# Autodesk Inventor assembly: Assembly1
(part 7 of 8)
## Named parameters: d38_d13 = 0 mm, d39_d14 = 0 mm, d40_d15 = 270 deg, d41_d16 = 0 mm, d42_d17 = 270 deg, d43_d3 = 25 deg, d44_d4 = -25 deg, d45_d5 = 25 deg, d46_d6 = -25 deg, d47_d2 = 0 mm, d48_d30 = 0 mm, d58_d13 = 0 mm, d59_d14 = 0 mm, d60_d15 = 270 deg, d61_d16 = 0 mm, d62_d17 = 270 deg, d63_d3 = 25 deg, d64_d4 = -25 deg, d65_d5 = 25 deg, d66_d6 = -25 deg, d67_d2 = 0 mm, d68_d30 = 0 mm, d78_d13 = 0 mm, d79_d14 = 0 mm, d80_d15 = 270 deg, d81_d16 = 0 mm, d82_d17 = 270 deg, d83_d3 = 25 deg, d84_d4 = -25 deg, d85_d5 = 25 deg, d86_d6 = -25 deg, d87_d2 = 0 mm, d88_d30 = 0 mm, d95_d13 = 0 mm, d96_d14 = 0 mm, d97_d15 = 270 deg, d98_d16 = 0 mm, d99_d17 = 270 deg, d100_d3 = 25 deg, d101_d4 = -25 deg, d102_d5 = 25 deg, d103_d6 = -25 deg, d104_d2 = 0 mm, d105_d30 = 0 mm, d112_d13 = 0 mm, d113_d14 = 0 mm, d114_d15 = 270 deg, d115_d16 = 0 mm, d116_d17 = 270 deg, d117_d3 = 25 deg, d118_d4 = -25 deg, d119_d5 = 25 deg, d120_d6 = -25 deg, d121_d2 = 0 mm, d122_d30 = 0 mm, d129_d13 = 0 mm, d130_d14 = 0 mm, d131_d15 = 270 deg, d132_d16 = 0 mm, d133_d17 = 270 deg, d134_d3 = 25 deg, d135_d4 = -25 deg, d136_d5 = 25 deg, d137_d6 = -25 deg, d138_d2 = 0 mm, d139_d30 = 0 mm, d146_d13 = 0 mm, d147_d14 = 0 mm, d148_d15 = 270 deg, d149_d16 = 0 mm, d150_d17 = 270 deg, d151_d3 = 25 deg, d152_d4 = -25 deg, d153_d5 = 25 deg, d154_d6 = -25 deg, d155_d2 = 0 mm, d156_d30 = 0 mm, d163_d13 = 0 mm, d164_d14 = 0 mm, d165_d15 = 270 deg, d166_d16 = 0 mm, d167_d17 = 270 deg, d168_d3 = 25 deg, d169_d4 = -25 deg, d170_d5 = 25 deg, d171_d6 = -25 deg, d172_d2 = 0 mm, d173_d30 = 0 mm, d180_d13 = 0 mm, d181_d14 = 0 mm, d182_d15 = 270 deg, d183_d16 = 0 mm, d184_d17 = 270 deg, d185_d3 = 25 deg, d186_d4 = -25 deg, d187_d5 = 25 deg, d188_d6 = -25 deg, d189_d2 = 0 mm, d190_d30 = 0 mm, d197_d13 = 0 mm, d198_d14 = 0 mm, d199_d15 = 270 deg, d200_d16 = 0 mm, d201_d17 = 270 deg, d202_d3 = 25 deg, d203_d4 = -25 deg, d204_d5 = 25 deg, d205_d6 = -25 deg, d206_d2 = 0 mm, d207_d30 = 0 mm, d214_d13 = 0 mm, d215_d14 = 0 mm, d216_d15 = 270 deg, d217_d16 = 0 mm, d218_d17 = 270 deg, d219_d3 = 25 deg, d220_d4 = -25 deg, d221_d5 = 25 deg, d222_d6 = -25 deg, d223_d2 = 0 mm, d224_d30 = 0 mm, d231_d13 = 0 mm, d232_d14 = 0 mm, d233_d15 = 270 deg, d234_d16 = 0 mm, d235_d17 = 270 deg, d236_d3 = 25 deg, d237_d4 = -25 deg, d238_d5 = 25 deg, d239_d6 = -25 deg, d240_d2 = 0 mm, d241_d30 = 0 mm, d248_d13 = 0 mm, d249_d14 = 0 mm, d250_d15 = 270 deg, d251_d16 = 0 mm, d252_d17 = 270 deg, d253_d3 = 25 deg, d254_d4 = -25 deg, d255_d5 = 25 deg, d256_d6 = -25 deg, d257_d2 = 0 mm, d258_d30 = 0 mm, d265_d13 = 0 mm, d266_d14 = 0 mm, d267_d15 = 270 deg, d268_d16 = 0 mm, d269_d17 = 270 deg, d270_d3 = 25 deg, d271_d4 = -25 deg, d272_d5 = 25 deg, d273_d6 = -25 deg, d274_d2 = 0 mm, d275_d30 = 0 mm, d318_d248_d13 = 0 mm, d319_d249_d14 = 0 mm, d320_d250_d15 = 270 deg, d321_d251_d16 = 0 mm, d322_d252_d17 = 270 deg, d323_d253_d3 = 25 deg, d324_d254_d4 = -25 deg, d325_d255_d5 = 25 deg, d326_d256_d6 = -25 deg, d327_d257_d2 = 0 mm, d328_d258_d30 = 0 mm, d335_d248_d13 = 0 mm, d336_d249_d14 = 0 mm, d337_d250_d15 = 270 deg, d338_d251_d16 = 0 mm, d339_d252_d17 = 270 deg, d340_d253_d3 = 25 deg, d341_d254_d4 = -25 deg, d342_d255_d5 = 25 deg, d343_d256_d6 = -25 deg, d344_d257_d2 = 0 mm, d345_d258_d30 = 0 mm, d352_d248_d13 = 0 mm, d353_d249_d14 = 0 mm, d354_d250_d15 = 270 deg, d355_d251_d16 = 0 mm, d356_d252_d17 = 270 deg, d357_d253_d3 = 25 deg, d358_d254_d4 = -25 deg, d359_d255_d5 = 25 deg, d360_d256_d6 = -25 deg, d361_d257_d2 = 0 mm, d362_d258_d30 = 0 mm, d369_d248_d13 = 0 mm, d370_d249_d14 = 0 mm, d371_d250_d15 = 270 deg, d372_d251_d16 = 0 mm, d373_d252_d17 = 270 deg, d374_d253_d3 = 25 deg, d375_d254_d4 = -25 deg, d376_d255_d5 = 25 deg, d377_d256_d6 = -25 deg, d378_d257_d2 = 0 mm, d379_d258_d30 = 0 mm, d386_d248_d13 = 0 mm, d387_d249_d14 = 0 mm, d388_d250_d15 = 270 deg, d389_d251_d16 = 0 mm, d390_d252_d17 = 270 deg, d391_d253_d3 = 25 deg, d392_d254_d4 = -25 deg, d393_d255_d5 = 25 deg, d394_d256_d6 = -25 deg, d395_d257_d2 = 0 mm, d396_d258_d30 = 0 mm, d418_d248_d13 = 0 mm, d419_d249_d14 = 0 mm, d420_d250_d15 = 270 deg, d421_d251_d16 = 0 mm, d422_d252_d17 = 270 deg, d423_d253_d3 = 25 deg, d424_d254_d4 = -25 deg, d425_d255_d5 = 25 deg, d426_d256_d6 = -25 deg, d427_d257_d2 = 0 mm, d428_d258_d30 = 0 mm, d435_d248_d13 = 0 mm, d436_d249_d14 = 0 mm, d437_d250_d15 = 270 deg, d438_d251_d16 = 0 mm, d439_d252_d17 = 270 deg, d440_d253_d3 = 25 deg, d441_d254_d4 = -25 deg, d442_d255_d5 = 25 deg, d443_d256_d6 = -25 deg, d444_d257_d2 = 0 mm, d445_d258_d30 = 0 mm, d452_d248_d13 = 0 mm, d453_d249_d14 = 0 mm, d454_d250_d15 = 270 deg, d455_d251_d16 = 0 mm, d456_d252_d17 = 270 deg, d457_d253_d3 = 25 deg, d458_d254_d4 = -25 deg, d459_d255_d5 = 25 deg, d460_d256_d6 = -25 deg, d461_d257_d2 = 0 mm, d462_d258_d30 = 0 mm, d469_d248_d13 = 0 mm, d470_d249_d14 = 0 mm, d471_d250_d15 = 270 deg, d472_d251_d16 = 0 mm, d473_d252_d17 = 270 deg, d474_d253_d3 = 25 deg, d475_d254_d4 = -25 deg, d476_d255_d5 = 25 deg, d477_d256_d6 = -25 deg, d478_d257_d2 = 0 mm, d479_d258_d30 = 0 mm, d498_d248_d13 = 0 mm, d499_d249_d14 = 0 mm, d500_d250_d15 = 270 deg, d501_d251_d16 = 0 mm, d502_d252_d17 = 270 deg, d503_d253_d3 = 25 deg, d504_d254_d4 = -25 deg, d505_d255_d5 = 25 deg, d506_d256_d6 = -25 deg, d507_d257_d2 = 0 mm, d508_d258_d30 = 0 mm, d515_d248_d13 = 0 mm, d516_d249_d14 = 0 mm, d517_d250_d15 = 270 deg, d518_d251_d16 = 0 mm, d519_d252_d17 = 270 deg, d520_d253_d3 = 25 deg, d521_d254_d4 = -25 deg, d522_d255_d5 = 25 deg, d523_d256_d6 = -25 deg, d524_d257_d2 = 0 mm, d525_d258_d30 = 0 mm, d532_d248_d13 = 0 mm, d533_d249_d14 = 0 mm, d534_d250_d15 = 270 deg, d535_d251_d16 = 0 mm, d536_d252_d17 = 270 deg, d537_d253_d3 = 25 deg, d538_d254_d4 = -25 deg, d539_d255_d5 = 25 deg, d540_d256_d6 = -25 deg, d541_d257_d2 = 0 mm, d542_d258_d30 = 0 mm, d549_d248_d13 = 0 mm, d550_d249_d14 = 0 mm, d551_d250_d15 = 270 deg, d552_d251_d16 = 0 mm, d553_d252_d17 = 270 deg, d554_d253_d3 = 25 deg, d555_d254_d4 = -25 deg, d556_d255_d5 = 25 deg, d557_d256_d6 = -25 deg, d558_d257_d2 = 0 mm, d559_d258_d30 = 0 mm, d566_d248_d13 = 0 mm, d567_d249_d14 = 0 mm, d568_d250_d15 = 270 deg, d569_d251_d16 = 0 mm, d570_d252_d17 = 270 deg, d571_d253_d3 = 25 deg, d572_d254_d4 = -25 deg, d573_d255_d5 = 25 deg, d574_d256_d6 = -25 deg, d575_d257_d2 = 0 mm, d576_d258_d30 = 0 mm, d583_d248_d13 = 0 mm, d584_d249_d14 = 0 mm, d585_d250_d15 = 270 deg, d586_d251_d16 = 0 mm, d587_d252_d17 = 270 deg, d588_d253_d3 = 25 deg, d589_d254_d4 = -25 deg, d590_d255_d5 = 25 deg, d591_d256_d6 = -25 deg, d592_d257_d2 = 0 mm, d593_d258_d30 = 0 mm, d600_d248_d13 = 0 mm, d601_d249_d14 = 0 mm, d602_d250_d15 = 270 deg, d603_d251_d16 = 0 mm, d604_d252_d17 = 270 deg, d605_d253_d3 = 25 deg, d606_d254_d4 = -25 deg, d607_d255_d5 = 25 deg, d608_d256_d6 = -25 deg, d609_d257_d2 = 0 mm, d610_d258_d30 = 0 mm, d617_d248_d13 = 0 mm, d618_d249_d14 = 0 mm, d619_d250_d15 = 270 deg, d620_d251_d16 = 0 mm, d621_d252_d17 = 270 deg, d622_d253_d3 = 25 deg, d623_d254_d4 = -25 deg, d624_d255_d5 = 25 deg, d625_d256_d6 = -25 deg, d626_d257_d2 = 0 mm, d627_d258_d30 = 0 mm, d634_d248_d13 = 0 mm, d635_d249_d14 = 0 mm, d636_d250_d15 = 270 deg, d637_d251_d16 = 0 mm, d638_d252_d17 = 270 deg, d639_d253_d3 = 25 deg, d640_d254_d4 = -25 deg, d641_d255_d5 = 25 deg, d642_d256_d6 = -25 deg, d643_d257_d2 = 0 mm, d644_d258_d30 = 0 mm, d651_d248_d13 = 0 mm, d652_d249_d14 = 0 mm, d653_d250_d15 = 270 deg, d654_d251_d16 = 0 mm, d655_d252_d17 = 270 deg, d656_d253_d3 = 25 deg, d657_d254_d4 = -25 deg, d658_d255_d5 = 25 deg, d659_d256_d6 = -25 deg, d660_d257_d2 = 0 mm, d661_d258_d30 = 0 mm, d668_d248_d13 = 0 mm, d669_d249_d14 = 0 mm, d670_d250_d15 = 270 deg, d671_d251_d16 = 0 mm, d672_d252_d17 = 270 deg, d673_d253_d3 = 25 deg, d674_d254_d4 = -25 deg, d675_d255_d5 = 25 deg, d676_d256_d6 = -25 deg, d677_d257_d2 = 0 mm, d678_d258_d30 = 0 mm, d685_d248_d13 = 0 mm, d686_d249_d14 = 0 mm, d687_d250_d15 = 270 deg, d688_d251_d16 = 0 mm, d689_d252_d17 = 270 deg, d690_d253_d3 = 25 deg, d691_d254_d4 = -25 deg, d692_d255_d5 = 25 deg, d693_d256_d6 = -25 deg, d694_d257_d2 = 0 mm, d695_d258_d30 = 0 mm, d702_d248_d13 = 0 mm, d703_d249_d14 = 0 mm, d704_d250_d15 = 270 deg, d705_d251_d16 = 0 mm, d706_d252_d17 = 270 deg, d707_d253_d3 = 25 deg, d708_d254_d4 = -25 deg, d709_d255_d5 = 25 deg, d710_d256_d6 = -25 deg, d711_d257_d2 = 0 mm, d712_d258_d30 = 0 mm, d758_d248_d13 = 0 mm, d759_d249_d14 = 0 mm, d760_d250_d15 = 270 deg, d761_d251_d16 = 0 mm, d762_d252_d17 = 270 deg, d763_d253_d3 = 25 deg, d764_d254_d4 = -25 deg, d765_d255_d5 = 25 deg, d766_d256_d6 = -25 deg, d767_d257_d2 = 0 mm, d768_d258_d30 = 0 mm, d775_d248_d13 = 0 mm, d776_d249_d14 = 0 mm, d777_d250_d15 = 270 deg, d778_d251_d16 = 0 mm, d779_d252_d17 = 270 deg, d780_d253_d3 = 25 deg, d781_d254_d4 = -25 deg, d782_d255_d5 = 25 deg, d783_d256_d6 = -25 deg, d784_d257_d2 = 0 mm, d785_d258_d30 = 0 mm, d792_d248_d13 = 0 mm, d793_d249_d14 = 0 mm, d794_d250_d15 = 270 deg, d795_d251_d16 = 0 mm, d796_d252_d17 = 270 deg, d797_d253_d3 = 25 deg, d798_d254_d4 = -25 deg, d799_d255_d5 = 25 deg, d800_d256_d6 = -25 deg, d801_d257_d2 = 0 mm, d802_d258_d30 = 0 mm, d809_d248_d13 = 0 mm, d810_d249_d14 = 0 mm, d811_d250_d15 = 270 deg, d812_d251_d16 = 0 mm, d813_d252_d17 = 270 deg, d814_d253_d3 = 25 deg, d815_d254_d4 = -25 deg, d816_d255_d5 = 25 deg, d817_d256_d6 = -25 deg, d818_d257_d2 = 0 mm, d819_d258_d30 = 0 mm, d826_d248_d13 = 0 mm, d827_d249_d14 = 0 mm, d828_d250_d15 = 270 deg, d829_d251_d16 = 0 mm, d830_d252_d17 = 270 deg, d831_d253_d3 = 25 deg, d832_d254_d4 = -25 deg, d833_d255_d5 = 25 deg, d834_d256_d6 = -25 deg, d835_d257_d2 = 0 mm, d836_d258_d30 = 0 mm, d843_d248_d13 = 0 mm, d844_d249_d14 = 0 mm, d845_d250_d15 = 270 deg, d846_d251_d16 = 0 mm, d847_d252_d17 = 270 deg, d848_d253_d3 = 25 deg, d849_d254_d4 = -25 deg, d850_d255_d5 = 25 deg, d851_d256_d6 = -25 deg, d852_d257_d2 = 0 mm, d853_d258_d30 = 0 mm, d860_d248_d13 = 0 mm, d861_d249_d14 = 0 mm, d862_d250_d15 = 270 deg, d863_d251_d16 = 0 mm, d864_d252_d17 = 270 deg, d865_d253_d3 = 25 deg, d866_d254_d4 = -25 deg, d867_d255_d5 = 25 deg, d868_d256_d6 = -25 deg, d869_d257_d2 = 0 mm, d870_d258_d30 = 0 mm, d877_d248_d13 = 0 mm, d878_d249_d14 = 0 mm, d879_d250_d15 = 270 deg, d880_d251_d16 = 0 mm, d881_d252_d17 = 270 deg, d882_d253_d3 = 25 deg, d883_d254_d4 = -25 deg, d884_d255_d5 = 25 deg, d885_d256_d6 = -25 deg, d886_d257_d2 = 0 mm, d887_d258_d30 = 0 mm, d918_d248_d13 = 0 mm, d919_d249_d14 = 0 mm, d920_d250_d15 = 270 deg, d921_d251_d16 = 0 mm, d922_d252_d17 = 270 deg, d923_d253_d3 = 25 deg, d924_d254_d4 = -25 deg, d925_d255_d5 = 25 deg, d926_d256_d6 = -25 deg, d927_d257_d2 = 0 mm, d928_d258_d30 = 0 mm, d935_d248_d13 = 0 mm, d936_d249_d14 = 0 mm, d937_d250_d15 = 270 deg, d938_d251_d16 = 0 mm, d939_d252_d17 = 270 deg, d940_d253_d3 = 25 deg, d941_d254_d4 = -25 deg, d942_d255_d5 = 25 deg, d943_d256_d6 = -25 deg, d944_d257_d2 = 0 mm, d945_d258_d30 = 0 mm, d952_d248_d13 = 0 mm, d953_d249_d14 = 0 mm, d954_d250_d15 = 270 deg, d955_d251_d16 = 0 mm, d956_d252_d17 = 270 deg, d957_d253_d3 = 25 deg, d958_d254_d4 = -25 deg, d959_d255_d5 = 25 deg, d960_d256_d6 = -25 deg, d961_d257_d2 = 0 mm, d962_d258_d30 = 0 mm, d986_d248_d13 = 0 mm, d987_d249_d14 = 0 mm, d988_d250_d15 = 270 deg, d989_d251_d16 = 0 mm, d990_d252_d17 = 270 deg, d991_d253_d3 = 25 deg, d992_d254_d4 = -25 deg, d993_d255_d5 = 25 deg, d994_d256_d6 = -25 deg, d995_d257_d2 = 0 mm, d996_d258_d30 = 0 mm, d1003_d248_d13 = 0 mm, d1004_d249_d14 = 0 mm, d1005_d250_d15 = 270 deg, d1006_d251_d16 = 0 mm, d1007_d252_d17 = 270 deg, d1008_d253_d3 = 25 deg, d1009_d254_d4 = -25 deg, d1010_d255_d5 = 25 deg, d1011_d256_d6 = -25 deg, d1012_d257_d2 = 0 mm, d1013_d258_d30 = 0 mm, d1037_d248_d13 = 0 mm, d1038_d249_d14 = 0 mm, d1039_d250_d15 = 270 deg, d1040_d251_d16 = 0 mm, d1041_d252_d17 = 270 deg, d1042_d253_d3 = 25 deg, d1043_d254_d4 = -25 deg, d1044_d255_d5 = 25 deg, d1045_d256_d6 = -25 deg, d1046_d257_d2 = 0 mm, d1047_d258_d30 = 0 mm, d1071_d248_d13 = 0 mm, d1072_d249_d14 = 0 mm, d1073_d250_d15 = 270 deg, d1074_d251_d16 = 0 mm, d1075_d252_d17 = 270 deg, d1076_d253_d3 = 25 deg, d1077_d254_d4 = -25 deg, d1078_d255_d5 = 25 deg, d1079_d256_d6 = -25 deg, d1080_d257_d2 = 0 mm, d1081_d258_d30 = 0 mm, d1105_d248_d13 = 0 mm, d1106_d249_d14 = 0 mm, d1107_d250_d15 = 270 deg, d1108_d251_d16 = 0 mm, d1109_d252_d17 = 270 deg, d1110_d253_d3 = 25 deg, d1111_d254_d4 = -25 deg, d1112_d255_d5 = 25 deg, d1113_d256_d6 = -25 deg, d1114_d257_d2 = 0 mm, d1115_d258_d30 = 0 mm, d1182_d248_d13 = 0 mm, d1183_d249_d14 = 0 mm, d1184_d250_d15 = 270 deg, d1185_d251_d16 = 0 mm, d1186_d252_d17 = 270 deg, d1187_d253_d3 = 25 deg, d1188_d254_d4 = -25 deg, d1189_d255_d5 = 25 deg, d1190_d256_d6 = -25 deg, d1191_d257_d2 = 0 mm, d1192_d258_d30 = 0 mm, d1199_d248_d13 = 0 mm, d1200_d249_d14 = 0 mm, d1201_d250_d15 = 270 deg, d1202_d251_d16 = 0 mm, d1203_d252_d17 = 270 deg, d1204_d253_d3 = 25 deg, d1205_d254_d4 = -25 deg, d1206_d255_d5 = 25 deg, d1207_d256_d6 = -25 deg, d1208_d257_d2 = 0 mm, d1209_d258_d30 = 0 mm, d1216_d248_d13 = 0 mm, d1217_d249_d14 = 0 mm, d1218_d250_d15 = 270 deg, d1219_d251_d16 = 0 mm, d1220_d252_d17 = 270 deg, d1221_d253_d3 = 25 deg, d1222_d254_d4 = -25 deg, d1223_d255_d5 = 25 deg, d1224_d256_d6 = -25 deg, d1225_d257_d2 = 0 mm, d1226_d258_d30 = 0 mm, d1233_d248_d13 = 0 mm, d1234_d249_d14 = 0 mm, d1235_d250_d15 = 270 deg, d1236_d251_d16 = 0 mm, d1237_d252_d17 = 270 deg, d1238_d253_d3 = 25 deg, d1239_d254_d4 = -25 deg, d1240_d255_d5 = 25 deg, d1241_d256_d6 = -25 deg, d1242_d257_d2 = 0 mm, d1243_d258_d30 = 0 mm, d1250_d248_d13 = 0 mm, d1251_d249_d14 = 0 mm, d1252_d250_d15 = 270 deg, d1253_d251_d16 = 0 mm, d1254_d252_d17 = 270 deg, d1255_d253_d3 = 25 deg, d1256_d254_d4 = -25 deg, d1257_d255_d5 = 25 deg, d1258_d256_d6 = -25 deg, d1259_d257_d2 = 0 mm, d1260_d258_d30 = 0 mm, d1267_d248_d13 = 0 mm, d1268_d249_d14 = 0 mm, d1269_d250_d15 = 270 deg, d1270_d251_d16 = 0 mm, d1271_d252_d17 = 270 deg, d1272_d253_d3 = 25 deg, d1273_d254_d4 = -25 deg, d1274_d255_d5 = 25 deg, d1275_d256_d6 = -25 deg, d1276_d257_d2 = 0 mm, d1277_d258_d30 = 0 mm, d1284_d248_d13 = 0 mm, d1285_d249_d14 = 0 mm, d1286_d250_d15 = 270 deg, d1287_d251_d16 = 0 mm, d1288_d252_d17 = 270 deg, d1289_d253_d3 = 25 deg, d1290_d254_d4 = -25 deg, d1291_d255_d5 = 25 deg, d1292_d256_d6 = -25 deg, d1293_d257_d2 = 0 mm, d1294_d258_d30 = 0 mm, d1301_d248_d13 = 0 mm, d1302_d249_d14 = 0 mm, d1303_d250_d15 = 270 deg, d1304_d251_d16 = 0 mm, d1305_d252_d17 = 270 deg, d1306_d253_d3 = 25 deg, d1307_d254_d4 = -25 deg, d1308_d255_d5 = 25 deg, d1309_d256_d6 = -25 deg, d1310_d257_d2 = 0 mm, d1311_d258_d30 = 0 mm, d1318_d248_d13 = 0 mm, d1319_d249_d14 = 0 mm, d1320_d250_d15 = 270 deg, d1321_d251_d16 = 0 mm, d1322_d252_d17 = 270 deg, d1323_d253_d3 = 25 deg, d1324_d254_d4 = -25 deg, d1325_d255_d5 = 25 deg, d1326_d256_d6 = -25 deg, d1327_d257_d2 = 0 mm, d1328_d258_d30 = 0 mm, d1335_d248_d13 = 0 mm, d1336_d249_d14 = 0 mm, d1337_d250_d15 = 270 deg, d1338_d251_d16 = 0 mm, d1339_d252_d17 = 270 deg, d1340_d253_d3 = 25 deg, d1341_d254_d4 = -25 deg, d1342_d255_d5 = 25 deg, d1343_d256_d6 = -25 deg, d1344_d257_d2 = 0 mm, d1345_d258_d30 = 0 mm, d1352_d248_d13 = 0 mm, d1353_d249_d14 = 0 mm, d1354_d250_d15 = 270 deg, d1355_d251_d16 = 0 mm, d1356_d252_d17 = 270 deg, d1357_d253_d3 = 25 deg, d1358_d254_d4 = -25 deg, d1359_d255_d5 = 25 deg, d1360_d256_d6 = -25 deg, d1361_d257_d2 = 0 mm, d1362_d258_d30 = 0 mm, d1403_d248_d13 = 0 mm, d1404_d249_d14 = 0 mm, d1405_d250_d15 = 270 deg, d1406_d251_d16 = 0 mm, d1407_d252_d17 = 270 deg, d1408_d253_d3 = 25 deg, d1409_d254_d4 = -25 deg, d1410_d255_d5 = 25 deg, d1411_d256_d6 = -25 deg, d1412_d257_d2 = 0 mm, d1413_d258_d30 = 0 mm, d1420_d248_d13 = 0 mm, d1421_d249_d14 = 0 mm, d1422_d250_d15 = 270 deg, d1423_d251_d16 = 0 mm, d1424_d252_d17 = 270 deg, d1425_d253_d3 = 25 deg, d1426_d254_d4 = -25 deg, d1427_d255_d5 = 25 deg, d1428_d256_d6 = -25 deg, d1429_d257_d2 = 0 mm, d1430_d258_d30 = 0 mm, d1437_d248_d13 = 0 mm, d1438_d249_d14 = 0 mm, d1439_d250_d15 = 270 deg, d1440_d251_d16 = 0 mm, d1441_d252_d17 = 270 deg, d1442_d253_d3 = 25 deg, d1443_d254_d4 = -25 deg, d1444_d255_d5 = 25 deg, d1445_d256_d6 = -25 deg, d1446_d257_d2 = 0 mm, d1447_d258_d30 = 0 mm, d1471_d248_d13 = 0 mm, d1472_d249_d14 = 0 mm, d1473_d250_d15 = 270 deg, d1474_d251_d16 = 0 mm, d1475_d252_d17 = 270 deg, d1476_d253_d3 = 25 deg, d1477_d254_d4 = -25 deg, d1478_d255_d5 = 25 deg, d1479_d256_d6 = -25 deg, d1480_d257_d2 = 0 mm, d1481_d258_d30 = 0 mm, d1488_d248_d13 = 0 mm, d1489_d249_d14 = 0 mm, d1490_d250_d15 = 270 deg, d1491_d251_d16 = 0 mm, d1492_d252_d17 = 270 deg, d1493_d253_d3 = 25 deg, d1494_d254_d4 = -25 deg, d1495_d255_d5 = 25 deg, d1496_d256_d6 = -25 deg, d1497_d257_d2 = 0 mm, d1498_d258_d30 = 0 mm, d1505_d248_d13 = 0 mm, d1506_d249_d14 = 0 mm, d1507_d250_d15 = 270 deg, d1508_d251_d16 = 0 mm, d1509_d252_d17 = 270 deg, d1510_d253_d3 = 25 deg, d1511_d254_d4 = -25 deg, d1512_d255_d5 = 25 deg, d1513_d256_d6 = -25 deg, d1514_d257_d2 = 0 mm, d1515_d258_d30 = 0 mm, d1522_d248_d13 = 0 mm, d1523_d249_d14 = 0 mm, d1524_d250_d15 = 270 deg, d1525_d251_d16 = 0 mm, d1526_d252_d17 = 270 deg, d1527_d253_d3 = 25 deg, d1528_d254_d4 = -25 deg, d1529_d255_d5 = 25 deg, d1530_d256_d6 = -25 deg, d1531_d257_d2 = 0 mm, d1532_d258_d30 = 0 mm, d1539_d248_d13 = 0 mm, d1540_d249_d14 = 0 mm, d1541_d250_d15 = 270 deg, d1542_d251_d16 = 0 mm, d1543_d252_d17 = 270 deg, d1544_d253_d3 = 25 deg, d1545_d254_d4 = -25 deg, d1546_d255_d5 = 25 deg, d1547_d256_d6 = -25 deg, d1548_d257_d2 = 0 mm, d1549_d258_d30 = 0 mm, d1556_d248_d13 = 0 mm, d1557_d249_d14 = 0 mm, d1558_d250_d15 = 270 deg, d1559_d251_d16 = 0 mm, d1560_d252_d17 = 270 deg, d1561_d253_d3 = 25 deg, d1562_d254_d4 = -25 deg, d1563_d255_d5 = 25 deg, d1564_d256_d6 = -25 deg, d1565_d257_d2 = 0 mm, d1566_d258_d30 = 0 mm, d1573_d248_d13 = 0 mm, d1574_d249_d14 = 0 mm, d1575_d250_d15 = 270 deg, d1576_d251_d16 = 0 mm, d1577_d252_d17 = 270 deg, d1578_d253_d3 = 25 deg, d1579_d254_d4 = -25 deg, d1580_d255_d5 = 25 deg, d1581_d256_d6 = -25 deg, d1582_d257_d2 = 0 mm, d1583_d258_d30 = 0 mm, d1590_d248_d13 = 0 mm, d1591_d249_d14 = 0 mm, d1592_d250_d15 = 270 deg, d1593_d251_d16 = 0 mm, d1594_d252_d17 = 270 deg, d1595_d253_d3 = 25 deg, d1596_d254_d4 = -25 deg, d1597_d255_d5 = 25 deg, d1598_d256_d6 = -25 deg, d1599_d257_d2 = 0 mm, d1600_d258_d30 = 0 mm, d1644_d248_d13 = 0 mm, d1645_d249_d14 = 0 mm, d1646_d250_d15 = 270 deg, d1647_d251_d16 = 0 mm, d1648_d252_d17 = 270 deg, d1649_d253_d3 = 25 deg, d1650_d254_d4 = -25 deg, d1651_d255_d5 = 25 deg, d1652_d256_d6 = -25 deg, d1653_d257_d2 = 0 mm, d1654_d258_d30 = 0 mm, d1661_d248_d13 = 0 mm, d1662_d249_d14 = 0 mm, d1663_d250_d15 = 270 deg, d1664_d251_d16 = 0 mm, d1665_d252_d17 = 270 deg, d1666_d253_d3 = 25 deg, d1667_d254_d4 = -25 deg, d1668_d255_d5 = 25 deg, d1669_d256_d6 = -25 deg, d1670_d257_d2 = 0 mm, d1671_d258_d30 = 0 mm, d1678_d248_d13 = 0 mm, d1679_d249_d14 = 0 mm, d1680_d250_d15 = 270 deg, d1681_d251_d16 = 0 mm, d1682_d252_d17 = 270 deg, d1683_d253_d3 = 25 deg, d1684_d254_d4 = -25 deg, d1685_d255_d5 = 25 deg, d1686_d256_d6 = -25 deg, d1687_d257_d2 = 0 mm, d1688_d258_d30 = 0 mm, d1695_d248_d13 = 0 mm, d1696_d249_d14 = 0 mm, d1697_d250_d15 = 270 deg, d1698_d251_d16 = 0 mm, d1699_d252_d17 = 270 deg, d1700_d253_d3 = 25 deg, d1701_d254_d4 = -25 deg, d1702_d255_d5 = 25 deg, d1703_d256_d6 = -25 deg, d1704_d257_d2 = 0 mm, d1705_d258_d30 = 0 mm, d1712_d248_d13 = 0 mm, d1713_d249_d14 = 0 mm, d1714_d250_d15 = 270 deg, d1715_d251_d16 = 0 mm, d1716_d252_d17 = 270 deg, d1717_d253_d3 = 25 deg, d1718_d254_d4 = -25 deg, d1719_d255_d5 = 25 deg, d1720_d256_d6 = -25 deg, d1721_d257_d2 = 0 mm, d1722_d258_d30 = 0 mm, d1729_d248_d13 = 0 mm, d1730_d249_d14 = 0 mm, d1731_d250_d15 = 270 deg, d1732_d251_d16 = 0 mm, d1733_d252_d17 = 270 deg, d1734_d253_d3 = 25 deg, d1735_d254_d4 = -25 deg, d1736_d255_d5 = 25 deg, d1737_d256_d6 = -25 deg, d1738_d257_d2 = 0 mm, d1739_d258_d30 = 0 mm, d1746_d248_d13 = 0 mm, d1747_d249_d14 = 0 mm, d1748_d250_d15 = 270 deg, d1749_d251_d16 = 0 mm, d1750_d252_d17 = 270 deg, d1751_d253_d3 = 25 deg, d1752_d254_d4 = -25 deg, d1753_d255_d5 = 25 deg, d1754_d256_d6 = -25 deg, d1755_d257_d2 = 0 mm, d1756_d258_d30 = 0 mm, d1763_d248_d13 = 0 mm, d1764_d249_d14 = 0 mm, d1765_d250_d15 = 270 deg, d1766_d251_d16 = 0 mm, d1767_d252_d17 = 270 deg, d1768_d253_d3 = 25 deg, d1769_d254_d4 = -25 deg, d1770_d255_d5 = 25 deg, d1771_d256_d6 = -25 deg, d1772_d257_d2 = 0 mm, d1773_d258_d30 = 0 mm, d1780_d248_d13 = 0 mm, d1781_d249_d14 = 0 mm, d1782_d250_d15 = 270 deg, d1783_d251_d16 = 0 mm, d1784_d252_d17 = 270 deg, d1785_d253_d3 = 25 deg, d1786_d254_d4 = -25 deg, d1787_d255_d5 = 25 deg, d1788_d256_d6 = -25 deg, d1789_d257_d2 = 0 mm, d1790_d258_d30 = 0 mm, d1824_d248_d13 = 0 mm, d1825_d249_d14 = 0 mm, d1826_d250_d15 = 270 deg, d1827_d251_d16 = 0 mm, d1828_d252_d17 = 270 deg, d1829_d253_d3 = 25 deg, d1830_d254_d4 = -25 deg, d1831_d255_d5 = 25 deg, d1832_d256_d6 = -25 deg, d1833_d257_d2 = 0 mm, d1834_d258_d30 = 0 mm, d1844_d248_d13 = 0 mm, d1845_d249_d14 = 0 mm, d1846_d250_d15 = 270 deg, d1847_d251_d16 = 0 mm, d1848_d252_d17 = 270 deg, d1849_d253_d3 = 25 deg, d1850_d254_d4 = -25 deg, d1851_d255_d5 = 25 deg, d1852_d256_d6 = -25 deg, d1853_d257_d2 = 0 mm, d1854_d258_d30 = 0 mm, d1861_d248_d13 = 0 mm, d1862_d249_d14 = 0 mm, d1863_d250_d15 = 270 deg, d1864_d251_d16 = 0 mm, d1865_d252_d17 = 270 deg, d1866_d253_d3 = 25 deg, d1867_d254_d4 = -25 deg, d1868_d255_d5 = 25 deg, d1869_d256_d6 = -25 deg, d1870_d257_d2 = 0 mm, d1871_d258_d30 = 0 mm, d1878_d248_d13 = 0 mm, d1879_d249_d14 = 0 mm, d1880_d250_d15 = 270 deg, d1881_d251_d16 = 0 mm, d1882_d252_d17 = 270 deg, d1883_d253_d3 = 25 deg, d1884_d254_d4 = -25 deg, d1885_d255_d5 = 25 deg, d1886_d256_d6 = -25 deg, d1887_d257_d2 = 0 mm, d1888_d258_d30 = 0 mm, d1895_d248_d13 = 0 mm, d1896_d249_d14 = 0 mm, d1897_d250_d15 = 270 deg, d1898_d251_d16 = 0 mm, d1899_d252_d17 = 270 deg, d1900_d253_d3 = 25 deg, d1901_d254_d4 = -25 deg, d1902_d255_d5 = 25 deg, d1903_d256_d6 = -25 deg, d1904_d257_d2 = 0 mm, d1905_d258_d30 = 0 mm, d1912_d248_d13 = 0 mm, d1913_d249_d14 = 0 mm, d1914_d250_d15 = 270 deg, d1915_d251_d16 = 0 mm, d1916_d252_d17 = 270 deg, d1917_d253_d3 = 25 deg, d1918_d254_d4 = -25 deg, d1919_d255_d5 = 25 deg, d1920_d256_d6 = -25 deg, d1921_d257_d2 = 0 mm, d1922_d258_d30 = 0 mm, d1929_d248_d13 = 0 mm, d1930_d249_d14 = 0 mm, d1931_d250_d15 = 270 deg, d1932_d251_d16 = 0 mm, d1933_d252_d17 = 270 deg, d1934_d253_d3 = 25 deg, d1935_d254_d4 = -25 deg, d1936_d255_d5 = 25 deg, d1937_d256_d6 = -25 deg, d1938_d257_d2 = 0 mm, d1939_d258_d30 = 0 mm, d1946_d248_d13 = 0 mm, d1947_d249_d14 = 0 mm, d1948_d250_d15 = 270 deg, d1949_d251_d16 = 0 mm, d1950_d252_d17 = 270 deg, d1951_d253_d3 = 25 deg, d1952_d254_d4 = -25 deg, d1953_d255_d5 = 25 deg, d1954_d256_d6 = -25 deg, d1955_d257_d2 = 0 mm, d1956_d258_d30 = 0 mm, d1963_d248_d13 = 0 mm, d1964_d249_d14 = 0 mm, d1965_d250_d15 = 270 deg, d1966_d251_d16 = 0 mm, d1967_d252_d17 = 270 deg, d1968_d253_d3 = 25 deg, d1969_d254_d4 = -25 deg, d1970_d255_d5 = 25 deg, d1971_d256_d6 = -25 deg, d1972_d257_d2 = 0 mm, d1973_d258_d30 = 0 mm, d1980_d248_d13 = 0 mm, d1981_d249_d14 = 0 mm, d1982_d250_d15 = 270 deg, d1983_d251_d16 = 0 mm, d1984_d252_d17 = 270 deg, d1985_d253_d3 = 25 deg, d1986_d254_d4 = -25 deg, d1987_d255_d5 = 25 deg, d1988_d256_d6 = -25 deg, d1989_d257_d2 = 0 mm, d1990_d258_d30 = 0 mm, d1997_d248_d13 = 0 mm, d1998_d249_d14 = 0 mm, d1999_d250_d15 = 270 deg, d2000_d251_d16 = 0 mm, d2001_d252_d17 = 270 deg, d2002_d253_d3 = 25 deg, d2003_d254_d4 = -25 deg, d2004_d255_d5 = 25 deg, d2005_d256_d6 = -25 deg, d2006_d257_d2 = 0 mm, d2007_d258_d30 = 0 mm, d2014_d248_d13 = 0 mm, d2015_d249_d14 = 0 mm, d2016_d250_d15 = 270 deg, d2017_d251_d16 = 0 mm, d2018_d252_d17 = 270 deg, d2019_d253_d3 = 25 deg, d2020_d254_d4 = -25 deg, d2021_d255_d5 = 25 deg, d2022_d256_d6 = -25 deg, d2023_d257_d2 = 0 mm, d2024_d258_d30 = 0 mm, d2064_d248_d13 = 0 mm, d2065_d249_d14 = 0 mm, d2066_d250_d15 = 270 deg, d2067_d251_d16 = 0 mm, d2068_d252_d17 = 270 deg, d2069_d253_d3 = 25 deg, d2070_d254_d4 = -25 deg, d2071_d255_d5 = 25 deg, d2072_d256_d6 = -25 deg, d2073_d257_d2 = 0 mm, d2074_d258_d30 = 0 mm, d2081_d248_d13 = 0 mm, d2082_d249_d14 = 0 mm, d2083_d250_d15 = 270 deg, d2084_d251_d16 = 0 mm, d2085_d252_d17 = 270 deg, d2086_d253_d3 = 25 deg, d2087_d254_d4 = -25 deg, d2088_d255_d5 = 25 deg, d2089_d256_d6 = -25 deg, d2090_d257_d2 = 0 mm, d2091_d258_d30 = 0 mm, d2098_d248_d13 = 0 mm, d2099_d249_d14 = 0 mm, d2100_d250_d15 = 270 deg, d2101_d251_d16 = 0 mm, d2102_d252_d17 = 270 deg, d2103_d253_d3 = 25 deg, d2104_d254_d4 = -25 deg, d2105_d255_d5 = 25 deg, d2106_d256_d6 = -25 deg, d2107_d257_d2 = 0 mm, d2108_d258_d30 = 0 mm, d2115_d248_d13 = 0 mm, d2116_d249_d14 = 0 mm, d2117_d250_d15 = 270 deg, d2118_d251_d16 = 0 mm, d2119_d252_d17 = 270 deg, d2120_d253_d3 = 25 deg, d2121_d254_d4 = -25 deg, d2122_d255_d5 = 25 deg, d2123_d256_d6 = -25 deg, d2124_d257_d2 = 0 mm, d2125_d258_d30 = 0 mm, d2132_d248_d13 = 0 mm, d2133_d249_d14 = 0 mm, d2134_d250_d15 = 270 deg, d2135_d251_d16 = 0 mm, d2136_d252_d17 = 270 deg, d2137_d253_d3 = 25 deg, d2138_d254_d4 = -25 deg, d2139_d255_d5 = 25 deg, d2140_d256_d6 = -25 deg, d2141_d257_d2 = 0 mm, d2142_d258_d30 = 0 mm, d2149_d248_d13 = 0 mm, d2150_d249_d14 = 0 mm, d2151_d250_d15 = 270 deg, d2152_d251_d16 = 0 mm, d2153_d252_d17 = 270 deg, d2154_d253_d3 = 25 deg, d2155_d254_d4 = -25 deg, d2156_d255_d5 = 25 deg, d2157_d256_d6 = -25 deg, d2158_d257_d2 = 0 mm, d2159_d258_d30 = 0 mm, d2166_d248_d13 = 0 mm, d2167_d249_d14 = 0 mm, d2168_d250_d15 = 270 deg, d2169_d251_d16 = 0 mm, d2170_d252_d17 = 270 deg, d2171_d253_d3 = 25 deg, d2172_d254_d4 = -25 deg, d2173_d255_d5 = 25 deg, d2174_d256_d6 = -25 deg, d2175_d257_d2 = 0 mm, d2176_d258_d30 = 0 mm, d2183_d248_d13 = 0 mm, d2184_d249_d14 = 0 mm, d2185_d250_d15 = 270 deg, d2186_d251_d16 = 0 mm, d2187_d252_d17 = 270 deg, d2188_d253_d3 = 25 deg, d2189_d254_d4 = -25 deg, d2190_d255_d5 = 25 deg, d2191_d256_d6 = -25 deg, d2192_d257_d2 = 0 mm, d2193_d258_d30 = 0 mm, d2200_d248_d13 = 0 mm, d2201_d249_d14 = 0 mm, d2202_d250_d15 = 270 deg, d2203_d251_d16 = 0 mm, d2204_d252_d17 = 270 deg, d2205_d253_d3 = 25 deg, d2206_d254_d4 = -25 deg, d2207_d255_d5 = 25 deg, d2208_d256_d6 = -25 deg, d2209_d257_d2 = 0 mm, d2210_d258_d30 = 0 mm, d2244_d248_d13 = 0 mm, d2245_d249_d14 = 0 mm, d2246_d250_d15 = 270 deg, d2247_d251_d16 = 0 mm, d2248_d252_d17 = 270 deg, d2249_d253_d3 = 25 deg, d2250_d254_d4 = -25 deg, d2251_d255_d5 = 25 deg, d2252_d256_d6 = -25 deg, d2253_d257_d2 = 0 mm, d2254_d258_d30 = 0 mm, d2261_d248_d13 = 0 mm, d2262_d249_d14 = 0 mm, d2263_d250_d15 = 270 deg, d2264_d251_d16 = 0 mm, d2265_d252_d17 = 270 deg, d2266_d253_d3 = 25 deg, d2267_d254_d4 = -25 deg, d2268_d255_d5 = 25 deg, d2269_d256_d6 = -25 deg, d2270_d257_d2 = 0 mm, d2271_d258_d30 = 0 mm, d2278_d248_d13 = 0 mm, d2279_d249_d14 = 0 mm, d2280_d250_d15 = 270 deg, d2281_d251_d16 = 0 mm, d2282_d252_d17 = 270 deg, d2283_d253_d3 = 25 deg, d2284_d254_d4 = -25 deg, d2285_d255_d5 = 25 deg, d2286_d256_d6 = -25 deg, d2287_d257_d2 = 0 mm, d2288_d258_d30 = 0 mm, d2295_d248_d13 = 0 mm, d2296_d249_d14 = 0 mm, d2297_d250_d15 = 270 deg, d2298_d251_d16 = 0 mm, d2299_d252_d17 = 270 deg, d2300_d253_d3 = 25 deg, d2301_d254_d4 = -25 deg, d2302_d255_d5 = 25 deg, d2303_d256_d6 = -25 deg, d2304_d257_d2 = 0 mm, d2305_d258_d30 = 0 mm, d2312_d248_d13 = 0 mm, d2313_d249_d14 = 0 mm, d2314_d250_d15 = 270 deg, d2315_d251_d16 = 0 mm, d2316_d252_d17 = 270 deg, d2317_d253_d3 = 25 deg, d2318_d254_d4 = -25 deg, d2319_d255_d5 = 25 deg, d2320_d256_d6 = -25 deg, d2321_d257_d2 = 0 mm, d2322_d258_d30 = 0 mm, d2329_d248_d13 = 0 mm, d2330_d249_d14 = 0 mm, d2331_d250_d15 = 270 deg, d2332_d251_d16 = 0 mm, d2333_d252_d17 = 270 deg, d2334_d253_d3 = 25 deg, d2335_d254_d4 = -25 deg, d2336_d255_d5 = 25 deg, d2337_d256_d6 = -25 deg, d2338_d257_d2 = 0 mm, d2339_d258_d30 = 0 mm, d2346_d248_d13 = 0 mm, d2347_d249_d14 = 0 mm, d2348_d250_d15 = 270 deg, d2349_d251_d16 = 0 mm, d2350_d252_d17 = 270 deg, d2351_d253_d3 = 25 deg, d2352_d254_d4 = -25 deg, d2353_d255_d5 = 25 deg, d2354_d256_d6 = -25 deg, d2355_d257_d2 = 0 mm, d2356_d258_d30 = 0 mm, d2363_d248_d13 = 0 mm, d2364_d249_d14 = 0 mm, d2365_d250_d15 = 270 deg, d2366_d251_d16 = 0 mm, d2367_d252_d17 = 270 deg, d2368_d253_d3 = 25 deg, d2369_d254_d4 = -25 deg, d2370_d255_d5 = 25 deg, d2371_d256_d6 = -25 deg, d2372_d257_d2 = 0 mm, d2373_d258_d30 = 0 mm, d2380_d248_d13 = 0 mm, d2381_d249_d14 = 0 mm, d2382_d250_d15 = 270 deg, d2383_d251_d16 = 0 mm, d2384_d252_d17 = 270 deg, d2385_d253_d3 = 25 deg, d2386_d254_d4 = -25 deg, d2387_d255_d5 = 25 deg, d2388_d256_d6 = -25 deg, d2389_d257_d2 = 0 mm, d2390_d258_d30 = 0 mm, d2397_d248_d13 = 0 mm, d2398_d249_d14 = 0 mm, d2399_d250_d15 = 270 deg, d2400_d251_d16 = 0 mm, d2401_d252_d17 = 270 deg, d2402_d253_d3 = 25 deg, d2403_d254_d4 = -25 deg, d2404_d255_d5 = 25 deg, d2405_d256_d6 = -25 deg, d2406_d257_d2 = 0 mm, d2407_d258_d30 = 0 mm, d2444_d248_d13 = 0 mm, d2445_d249_d14 = 0 mm, d2446_d250_d15 = 270 deg, d2447_d251_d16 = 0 mm, d2448_d252_d17 = 270 deg, d2449_d253_d3 = 25 deg, d2450_d254_d4 = -25 deg, d2451_d255_d5 = 25 deg, d2452_d256_d6 = -25 deg, d2453_d257_d2 = 0 mm, d2454_d258_d30 = 0 mm, d2461_d248_d13 = 0 mm, d2462_d249_d14 = 0 mm, d2463_d250_d15 = 270 deg, d2464_d251_d16 = 0 mm, d2465_d252_d17 = 270 deg, d2466_d253_d3 = 25 deg, d2467_d254_d4 = -25 deg, d2468_d255_d5 = 25 deg, d2469_d256_d6 = -25 deg, d2470_d257_d2 = 0 mm, d2471_d258_d30 = 0 mm, d2478_d248_d13 = 0 mm, d2479_d249_d14 = 0 mm, d2480_d250_d15 = 270 deg, d2481_d251_d16 = 0 mm, d2482_d252_d17 = 270 deg, d2483_d253_d3 = 25 deg, d2484_d254_d4 = -25 deg, d2485_d255_d5 = 25 deg, d2486_d256_d6 = -25 deg, d2487_d257_d2 = 0 mm, d2488_d258_d30 = 0 mm, d2495_d248_d13 = 0 mm, d2496_d249_d14 = 0 mm, d2497_d250_d15 = 270 deg, d2498_d251_d16 = 0 mm, d2499_d252_d17 = 270 deg, d2500_d253_d3 = 25 deg, d2501_d254_d4 = -25 deg, d2502_d255_d5 = 25 deg, d2503_d256_d6 = -25 deg, d2504_d257_d2 = 0 mm, d2505_d258_d30 = 0 mm, d2512_d248_d13 = 0 mm, d2513_d249_d14 = 0 mm, d2514_d250_d15 = 270 deg, d2515_d251_d16 = 0 mm, d2516_d252_d17 = 270 deg, d2517_d253_d3 = 25 deg, d2518_d254_d4 = -25 deg, d2519_d255_d5 = 25 deg, d2520_d256_d6 = -25 deg, d2521_d257_d2 = 0 mm, d2522_d258_d30 = 0 mm, d2529_d248_d13 = 0 mm, d2530_d249_d14 = 0 mm, d2531_d250_d15 = 270 deg, d2532_d251_d16 = 0 mm, d2533_d252_d17 = 270 deg, d2534_d253_d3 = 25 deg, d2535_d254_d4 = -25 deg, d2536_d255_d5 = 25 deg, d2537_d256_d6 = -25 deg, d2538_d257_d2 = 0 mm, d2539_d258_d30 = 0 mm, d2546_d248_d13 = 0 mm, d2547_d249_d14 = 0 mm, d2548_d250_d15 = 270 deg, d2549_d251_d16 = 0 mm, d2550_d252_d17 = 270 deg, d2551_d253_d3 = 25 deg, d2552_d254_d4 = -25 deg, d2553_d255_d5 = 25 deg, d2554_d256_d6 = -25 deg, d2555_d257_d2 = 0 mm, d2556_d258_d30 = 0 mm, d2584_d248_d13 = 0 mm, d2585_d249_d14 = 0 mm, d2586_d250_d15 = 270 deg, d2587_d251_d16 = 0 mm, d2588_d252_d17 = 270 deg, d2589_d253_d3 = 25 deg, d2590_d254_d4 = -25 deg, d2591_d255_d5 = 25 deg, d2592_d256_d6 = -25 deg, d2593_d257_d2 = 0 mm, d2594_d258_d30 = 0 mm, d2601_d248_d13 = 0 mm, d2602_d249_d14 = 0 mm, d2603_d250_d15 = 270 deg, d2604_d251_d16 = 0 mm, d2605_d252_d17 = 270 deg, d2606_d253_d3 = 25 deg, d2607_d254_d4 = -25 deg, d2608_d255_d5 = 25 deg, d2609_d256_d6 = -25 deg, d2610_d257_d2 = 0 mm, d2611_d258_d30 = 0 mm, d2618_d248_d13 = 0 mm, d2619_d249_d14 = 0 mm, d2620_d250_d15 = 270 deg, d2621_d251_d16 = 0 mm, d2622_d252_d17 = 270 deg, d2623_d253_d3 = 25 deg, d2624_d254_d4 = -25 deg, d2625_d255_d5 = 25 deg, d2626_d256_d6 = -25 deg, d2627_d257_d2 = 0 mm, d2628_d258_d30 = 0 mm, d2635_d248_d13 = 0 mm, d2636_d249_d14 = 0 mm, d2637_d250_d15 = 270 deg, d2638_d251_d16 = 0 mm, d2639_d252_d17 = 270 deg, d2640_d253_d3 = 25 deg, d2641_d254_d4 = -25 deg, d2642_d255_d5 = 25 deg, d2643_d256_d6 = -25 deg, d2644_d257_d2 = 0 mm, d2645_d258_d30 = 0 mm, d2652_d248_d13 = 0 mm, d2653_d249_d14 = 0 mm, d2654_d250_d15 = 270 deg, d2655_d251_d16 = 0 mm, d2656_d252_d17 = 270 deg, d2657_d253_d3 = 25 deg, d2658_d254_d4 = -25 deg, d2659_d255_d5 = 25 deg, d2660_d256_d6 = -25 deg, d2661_d257_d2 = 0 mm, d2662_d258_d30 = 0 mm, d2669_d248_d13 = 0 mm, d2670_d249_d14 = 0 mm, d2671_d250_d15 = 270 deg, d2672_d251_d16 = 0 mm, d2673_d252_d17 = 270 deg, d2674_d253_d3 = 25 deg, d2675_d254_d4 = -25 deg, d2676_d255_d5 = 25 deg, d2677_d256_d6 = -25 deg, d2678_d257_d2 = 0 mm, d2679_d258_d30 = 0 mm, d2686_d248_d13 = 0 mm, d2687_d249_d14 = 0 mm, d2688_d250_d15 = 270 deg, d2689_d251_d16 = 0 mm, d2690_d252_d17 = 270 deg, d2691_d253_d3 = 25 deg, d2692_d254_d4 = -25 deg, d2693_d255_d5 = 25 deg, d2694_d256_d6 = -25 deg, d2695_d257_d2 = 0 mm, d2696_d258_d30 = 0 mm, d2703_d248_d13 = 0 mm, d2704_d249_d14 = 0 mm, d2705_d250_d15 = 270 deg, d2706_d251_d16 = 0 mm, d2707_d252_d17 = 270 deg, d2708_d253_d3 = 25 deg, d2709_d254_d4 = -25 deg, d2710_d255_d5 = 25 deg, d2711_d256_d6 = -25 deg, d2712_d257_d2 = 0 mm, d2713_d258_d30 = 0 mm, d2743_d248_d13 = 0 mm, d2744_d249_d14 = 0 mm, d2745_d250_d15 = 270 deg, d2746_d251_d16 = 0 mm, d2747_d252_d17 = 270 deg, d2748_d253_d3 = 25 deg, d2749_d254_d4 = -25 deg, d2750_d255_d5 = 25 deg, d2751_d256_d6 = -25 deg, d2752_d257_d2 = 0 mm, d2753_d258_d30 = 0 mm, d2760_d248_d13 = 0 mm, d2761_d249_d14 = 0 mm, d2762_d250_d15 = 270 deg, d2763_d251_d16 = 0 mm, d2764_d252_d17 = 270 deg, d2765_d253_d3 = 25 deg, d2766_d254_d4 = -25 deg, d2767_d255_d5 = 25 deg, d2768_d256_d6 = -25 deg, d2769_d257_d2 = 0 mm, d2770_d258_d30 = 0 mm, d2777_d248_d13 = 0 mm, d2778_d249_d14 = 0 mm, d2779_d250_d15 = 270 deg, d2780_d251_d16 = 0 mm, d2781_d252_d17 = 270 deg, d2782_d253_d3 = 25 deg, d2783_d254_d4 = -25 deg, d2784_d255_d5 = 25 deg, d2785_d256_d6 = -25 deg, d2786_d257_d2 = 0 mm, d2787_d258_d30 = 0 mm, d2794_d248_d13 = 0 mm, d2795_d249_d14 = 0 mm, d2796_d250_d15 = 270 deg, d2797_d251_d16 = 0 mm, d2798_d252_d17 = 270 deg, d2799_d253_d3 = 25 deg, d2800_d254_d4 = -25 deg, d2801_d255_d5 = 25 deg, d2802_d256_d6 = -25 deg, d2803_d257_d2 = 0 mm, d2804_d258_d30 = 0 mm, d2811_d248_d13 = 0 mm, d2812_d249_d14 = 0 mm, d2813_d250_d15 = 270 deg, d2814_d251_d16 = 0 mm, d2815_d252_d17 = 270 deg, d2816_d253_d3 = 25 deg, d2817_d254_d4 = -25 deg, d2818_d255_d5 = 25 deg, d2819_d256_d6 = -25 deg, d2820_d257_d2 = 0 mm, d2821_d258_d30 = 0 mm, d2828_d248_d13 = 0 mm, d2829_d249_d14 = 0 mm, d2830_d250_d15 = 270 deg, d2831_d251_d16 = 0 mm, d2832_d252_d17 = 270 deg, d2833_d253_d3 = 25 deg, d2834_d254_d4 = -25 deg, d2835_d255_d5 = 25 deg, d2836_d256_d6 = -25 deg, d2837_d257_d2 = 0 mm, d2838_d258_d30 = 0 mm, d2863_d248_d13 = 0 mm, d2864_d249_d14 = 0 mm, d2865_d250_d15 = 270 deg, d2866_d251_d16 = 0 mm, d2867_d252_d17 = 270 deg, d2868_d253_d3 = 25 deg, d2869_d254_d4 = -25 deg, d2870_d255_d5 = 25 deg, d2871_d256_d6 = -25 deg, d2872_d257_d2 = 0 mm, d2873_d258_d30 = 0 mm, d2880_d248_d13 = 0 mm, d2881_d249_d14 = 0 mm, d2882_d250_d15 = 270 deg, d2883_d251_d16 = 0 mm, d2884_d252_d17 = 270 deg, d2885_d253_d3 = 25 deg, d2886_d254_d4 = -25 deg, d2887_d255_d5 = 25 deg, d2888_d256_d6 = -25 deg, d2889_d257_d2 = 0 mm, d2890_d258_d30 = 0 mm, d2897_d248_d13 = 0 mm, d2898_d249_d14 = 0 mm, d2899_d250_d15 = 270 deg, d2900_d251_d16 = 0 mm, d2901_d252_d17 = 270 deg, d2902_d253_d3 = 25 deg, d2903_d254_d4 = -25 deg, d2904_d255_d5 = 25 deg, d2905_d256_d6 = -25 deg, d2906_d257_d2 = 0 mm, d2907_d258_d30 = 0 mm, d2914_d248_d13 = 0 mm, d2915_d249_d14 = 0 mm, d2916_d250_d15 = 270 deg, d2917_d251_d16 = 0 mm, d2918_d252_d17 = 270 deg, d2919_d253_d3 = 25 deg, d2920_d254_d4 = -25 deg, d2921_d255_d5 = 25 deg, d2922_d256_d6 = -25 deg, d2923_d257_d2 = 0 mm, d2924_d258_d30 = 0 mm, d2931_d248_d13 = 0 mm, d2932_d249_d14 = 0 mm, d2933_d250_d15 = 270 deg, d2934_d251_d16 = 0 mm, d2935_d252_d17 = 270 deg, d2936_d253_d3 = 25 deg, d2937_d254_d4 = -25 deg, d2938_d255_d5 = 25 deg, d2939_d256_d6 = -25 deg, d2940_d257_d2 = 0 mm, d2941_d258_d30 = 0 mm, d2948_d248_d13 = 0 mm, d2949_d249_d14 = 0 mm, d2950_d250_d15 = 270 deg, d2951_d251_d16 = 0 mm, d2952_d252_d17 = 270 deg, d2953_d253_d3 = 25 deg, d2954_d254_d4 = -25 deg, d2955_d255_d5 = 25 deg, d2956_d256_d6 = -25 deg, d2957_d257_d2 = 0 mm, d2958_d258_d30 = 0 mm, d2983_d248_d13 = 0 mm, d2984_d249_d14 = 0 mm, d2985_d250_d15 = 270 deg, d2986_d251_d16 = 0 mm, d2987_d252_d17 = 270 deg, d2988_d253_d3 = 25 deg, d2989_d254_d4 = -25 deg, d2990_d255_d5 = 25 deg, d2991_d256_d6 = -25 deg, d2992_d257_d2 = 0 mm, d2993_d258_d30 = 0 mm, d3000_d248_d13 = 0 mm, d3001_d249_d14 = 0 mm, d3002_d250_d15 = 270 deg, d3003_d251_d16 = 0 mm, d3004_d252_d17 = 270 deg, d3005_d253_d3 = 25 deg, d3006_d254_d4 = -25 deg, d3007_d255_d5 = 25 deg, d3008_d256_d6 = -25 deg, d3009_d257_d2 = 0 mm, d3010_d258_d30 = 0 mm, d3017_d248_d13 = 0 mm, d3018_d249_d14 = 0 mm, d3019_d250_d15 = 270 deg, d3020_d251_d16 = 0 mm, d3021_d252_d17 = 270 deg, d3022_d253_d3 = 25 deg, d3023_d254_d4 = -25 deg, d3024_d255_d5 = 25 deg, d3025_d256_d6 = -25 deg, d3026_d257_d2 = 0 mm, d3027_d258_d30 = 0 mm, d3034_d248_d13 = 0 mm, d3035_d249_d14 = 0 mm, d3036_d250_d15 = 270 deg, d3037_d251_d16 = 0 mm, d3038_d252_d17 = 270 deg, d3039_d253_d3 = 25 deg, d3040_d254_d4 = -25 deg, d3041_d255_d5 = 25 deg, d3042_d256_d6 = -25 deg, d3043_d257_d2 = 0 mm, d3044_d258_d30 = 0 mm, d3051_d248_d13 = 0 mm, d3052_d249_d14 = 0 mm, d3053_d250_d15 = 270 deg, d3054_d251_d16 = 0 mm, d3055_d252_d17 = 270 deg, d3056_d253_d3 = 25 deg, d3057_d254_d4 = -25 deg, d3058_d255_d5 = 25 deg, d3059_d256_d6 = -25 deg, d3060_d257_d2 = 0 mm, d3061_d258_d30 = 0 mm, d3083_d248_d13 = 0 mm, d3084_d249_d14 = 0 mm, d3085_d250_d15 = 270 deg, d3086_d251_d16 = 0 mm, d3087_d252_d17 = 270 deg, d3088_d253_d3 = 25 deg, d3089_d254_d4 = -25 deg, d3090_d255_d5 = 25 deg, d3091_d256_d6 = -25 deg, d3092_d257_d2 = 0 mm, d3093_d258_d30 = 0 mm, d3100_d248_d13 = 0 mm, d3101_d249_d14 = 0 mm, d3102_d250_d15 = 270 deg, d3103_d251_d16 = 0 mm, d3104_d252_d17 = 270 deg, d3105_d253_d3 = 25 deg, d3106_d254_d4 = -25 deg, d3107_d255_d5 = 25 deg, d3108_d256_d6 = -25 deg, d3109_d257_d2 = 0 mm, d3110_d258_d30 = 0 mm, d3117_d248_d13 = 0 mm, d3118_d249_d14 = 0 mm, d3119_d250_d15 = 270 deg, d3120_d251_d16 = 0 mm, d3121_d252_d17 = 270 deg, d3122_d253_d3 = 25 deg, d3123_d254_d4 = -25 deg, d3124_d255_d5 = 25 deg, d3125_d256_d6 = -25 deg, d3126_d257_d2 = 0 mm, d3127_d258_d30 = 0 mm, d3134_d248_d13 = 0 mm, d3135_d249_d14 = 0 mm, d3136_d250_d15 = 270 deg, d3137_d251_d16 = 0 mm, d3138_d252_d17 = 270 deg, d3139_d253_d3 = 25 deg, d3140_d254_d4 = -25 deg, d3141_d255_d5 = 25 deg, d3142_d256_d6 = -25 deg, d3143_d257_d2 = 0 mm, d3144_d258_d30 = 0 mm, d3151_d248_d13 = 0 mm, d3152_d249_d14 = 0 mm, d3153_d250_d15 = 270 deg, d3154_d251_d16 = 0 mm, d3155_d252_d17 = 270 deg, d3156_d253_d3 = 25 deg, d3157_d254_d4 = -25 deg, d3158_d255_d5 = 25 deg, d3159_d256_d6 = -25 deg, d3160_d257_d2 = 0 mm, d3161_d258_d30 = 0 mm, d3183_d248_d13 = 0 mm, d3184_d249_d14 = 0 mm, d3185_d250_d15 = 270 deg, d3186_d251_d16 = 0 mm, d3187_d252_d17 = 270 deg, d3188_d253_d3 = 25 deg, d3189_d254_d4 = -25 deg, d3190_d255_d5 = 25 deg, d3191_d256_d6 = -25 deg, d3192_d257_d2 = 0 mm, d3193_d258_d30 = 0 mm, d3200_d248_d13 = 0 mm, d3201_d249_d14 = 0 mm, d3202_d250_d15 = 270 deg, d3203_d251_d16 = 0 mm, d3204_d252_d17 = 270 deg, d3205_d253_d3 = 25 deg, d3206_d254_d4 = -25 deg, d3207_d255_d5 = 25 deg, d3208_d256_d6 = -25 deg, d3209_d257_d2 = 0 mm, d3210_d258_d30 = 0 mm, d3217_d248_d13 = 0 mm, d3218_d249_d14 = 0 mm, d3219_d250_d15 = 270 deg, d3220_d251_d16 = 0 mm, d3221_d252_d17 = 270 deg, d3222_d253_d3 = 25 deg, d3223_d254_d4 = -25 deg, d3224_d255_d5 = 25 deg, d3225_d256_d6 = -25 deg, d3226_d257_d2 = 0 mm, d3227_d258_d30 = 0 mm, d3234_d248_d13 = 0 mm, d3235_d249_d14 = 0 mm, d3236_d250_d15 = 270 deg, d3237_d251_d16 = 0 mm, d3238_d252_d17 = 270 deg, d3239_d253_d3 = 25 deg, d3240_d254_d4 = -25 deg, d3241_d255_d5 = 25 deg, d3242_d256_d6 = -25 deg, d3243_d257_d2 = 0 mm, d3244_d258_d30 = 0 mm, d3263_d248_d13 = 0 mm, d3264_d249_d14 = 0 mm, d3265_d250_d15 = 270 deg, d3266_d251_d16 = 0 mm, d3267_d252_d17 = 270 deg, d3268_d253_d3 = 25 deg, d3269_d254_d4 = -25 deg, d3270_d255_d5 = 25 deg, d3271_d256_d6 = -25 deg, d3272_d257_d2 = 0 mm, d3273_d258_d30 = 0 mm, d3280_d248_d13 = 0 mm, d3281_d249_d14 = 0 mm, d3282_d250_d15 = 270 deg, d3283_d251_d16 = 0 mm, d3284_d252_d17 = 270 deg, d3285_d253_d3 = 25 deg, d3286_d254_d4 = -25 deg, d3287_d255_d5 = 25 deg, d3288_d256_d6 = -25 deg, d3289_d257_d2 = 0 mm, d3290_d258_d30 = 0 mm, d3297_d248_d13 = 0 mm, d3298_d249_d14 = 0 mm, d3299_d250_d15 = 270 deg, d3300_d251_d16 = 0 mm, d3301_d252_d17 = 270 deg, d3302_d253_d3 = 25 deg, d3303_d254_d4 = -25 deg, d3304_d255_d5 = 25 deg, d3305_d256_d6 = -25 deg, d3306_d257_d2 = 0 mm, d3307_d258_d30 = 0 mm, d3314_d248_d13 = 0 mm, d3315_d249_d14 = 0 mm, d3316_d250_d15 = 270 deg, d3317_d251_d16 = 0 mm, d3318_d252_d17 = 270 deg, d3319_d253_d3 = 25 deg, d3320_d254_d4 = -25 deg, d3321_d255_d5 = 25 deg, d3322_d256_d6 = -25 deg, d3323_d257_d2 = 0 mm, d3324_d258_d30 = 0 mm, d3331_d248_d13 = 0 mm, d3332_d249_d14 = 0 mm, d3333_d250_d15 = 270 deg, d3334_d251_d16 = 0 mm, d3335_d252_d17 = 270 deg, d3336_d253_d3 = 25 deg, d3337_d254_d4 = -25 deg, d3338_d255_d5 = 25 deg, d3339_d256_d6 = -25 deg, d3340_d257_d2 = 0 mm, d3341_d258_d30 = 0 mm, d3348_d248_d13 = 0 mm, d3349_d249_d14 = 0 mm, d3350_d250_d15 = 270 deg, d3351_d251_d16 = 0 mm, d3352_d252_d17 = 270 deg, d3353_d253_d3 = 25 deg, d3354_d254_d4 = -25 deg, d3355_d255_d5 = 25 deg, d3356_d256_d6 = -25 deg, d3357_d257_d2 = 0 mm, d3358_d258_d30 = 0 mm, d3365_d248_d13 = 0 mm, d3366_d249_d14 = 0 mm, d3367_d250_d15 = 270 deg, d3368_d251_d16 = 0 mm, d3369_d252_d17 = 270 deg, d3370_d253_d3 = 25 deg, d3371_d254_d4 = -25 deg, d3372_d255_d5 = 25 deg, d3373_d256_d6 = -25 deg, d3374_d257_d2 = 0 mm, d3375_d258_d30 = 0 mm, d3403_d248_d13 = 0 mm, d3404_d249_d14 = 0 mm, d3405_d250_d15 = 270 deg, d3406_d251_d16 = 0 mm, d3407_d252_d17 = 270 deg, d3408_d253_d3 = 25 deg, d3409_d254_d4 = -25 deg, d3410_d255_d5 = 25 deg, d3411_d256_d6 = -25 deg, d3412_d257_d2 = 0 mm, d3413_d258_d30 = 0 mm, d3420_d248_d13 = 0 mm, d3421_d249_d14 = 0 mm, d3422_d250_d15 = 270 deg, d3423_d251_d16 = 0 mm, d3424_d252_d17 = 270 deg, d3425_d253_d3 = 25 deg, d3426_d254_d4 = -25 deg, d3427_d255_d5 = 25 deg, d3428_d256_d6 = -25 deg, d3429_d257_d2 = 0 mm, d3430_d258_d30 = 0 mm, d3437_d248_d13 = 0 mm, d3438_d249_d14 = 0 mm, d3439_d250_d15 = 270 deg, d3440_d251_d16 = 0 mm, d3441_d252_d17 = 270 deg, d3442_d253_d3 = 25 deg, d3443_d254_d4 = -25 deg, d3444_d255_d5 = 25 deg, d3445_d256_d6 = -25 deg, d3446_d257_d2 = 0 mm, d3447_d258_d30 = 0 mm, d3454_d248_d13 = 0 mm, d3455_d249_d14 = 0 mm, d3456_d250_d15 = 270 deg, d3457_d251_d16 = 0 mm, d3458_d252_d17 = 270 deg, d3459_d253_d3 = 25 deg, d3460_d254_d4 = -25 deg, d3461_d255_d5 = 25 deg, d3462_d256_d6 = -25 deg, d3463_d257_d2 = 0 mm, d3464_d258_d30 = 0 mm, d3471_d248_d13 = 0 mm, d3472_d249_d14 = 0 mm, d3473_d250_d15 = 270 deg, d3474_d251_d16 = 0 mm, d3475_d252_d17 = 270 deg, d3476_d253_d3 = 25 deg, d3477_d254_d4 = -25 deg, d3478_d255_d5 = 25 deg, d3479_d256_d6 = -25 deg, d3480_d257_d2 = 0 mm, d3481_d258_d30 = 0 mm, d3488_d248_d13 = 0 mm, d3489_d249_d14 = 0 mm, d3490_d250_d15 = 270 deg, d3491_d251_d16 = 0 mm, d3492_d252_d17 = 270 deg, d3493_d253_d3 = 25 deg, d3494_d254_d4 = -25 deg, d3495_d255_d5 = 25 deg, d3496_d256_d6 = -25 deg, d3497_d257_d2 = 0 mm, d3498_d258_d30 = 0 mm, d3505_d248_d13 = 0 mm, d3506_d249_d14 = 0 mm, d3507_d250_d15 = 270 deg, d3508_d251_d16 = 0 mm, d3509_d252_d17 = 270 deg, d3510_d253_d3 = 25 deg, d3511_d254_d4 = -25 deg, d3512_d255_d5 = 25 deg, d3513_d256_d6 = -25 deg, d3514_d257_d2 = 0 mm, d3515_d258_d30 = 0 mm, d3522_d248_d13 = 0 mm, d3523_d249_d14 = 0 mm, d3524_d250_d15 = 270 deg, d3525_d251_d16 = 0 mm, d3526_d252_d17 = 270 deg, d3527_d253_d3 = 25 deg, d3528_d254_d4 = -25 deg, d3529_d255_d5 = 25 deg, d3530_d256_d6 = -25 deg, d3531_d257_d2 = 0 mm, d3532_d258_d30 = 0 mm, d3539_d248_d13 = 0 mm, d3540_d249_d14 = 0 mm, d3541_d250_d15 = 270 deg, d3542_d251_d16 = 0 mm, d3543_d252_d17 = 270 deg, d3544_d253_d3 = 25 deg, d3545_d254_d4 = -25 deg, d3546_d255_d5 = 25 deg, d3547_d256_d6 = -25 deg, d3548_d257_d2 = 0 mm, d3549_d258_d30 = 0 mm, d3617_d952_d248_d13 = 0 mm, d3618_d953_d249_d14 = 0 mm, d3619_d954_d250_d15 = 270 deg, d3620_d955_d251_d16 = 0 mm, d3621_d956_d252_d17 = 270 deg, d3622_d957_d253_d3 = 25 deg, d3623_d958_d254_d4 = -25 deg, d3624_d959_d255_d5 = 25 deg, d3625_d960_d256_d6 = -25 deg, d3626_d961_d257_d2 = 0 mm, d3627_d962_d258_d30 = 0 mm, d3637_d952_d248_d13 = 0 mm, d3638_d953_d249_d14 = 0 mm, d3639_d954_d250_d15 = 270 deg, d3640_d955_d251_d16 = 0 mm, d3641_d956_d252_d17 = 270 deg, d3642_d957_d253_d3 = 25 deg, d3643_d958_d254_d4 = -25 deg, d3644_d959_d255_d5 = 25 deg, d3645_d960_d256_d6 = -25 deg, d3646_d961_d257_d2 = 0 mm, d3647_d962_d258_d30 = 0 mm, d3654_d952_d248_d13 = 0 mm, d3655_d953_d249_d14 = 0 mm, d3656_d954_d250_d15 = 270 deg, d3657_d955_d251_d16 = 0 mm, d3658_d956_d252_d17 = 270 deg, d3659_d957_d253_d3 = 25 deg, d3660_d958_d254_d4 = -25 deg, d3661_d959_d255_d5 = 25 deg, d3662_d960_d256_d6 = -25 deg, d3663_d961_d257_d2 = 0 mm, d3664_d962_d258_d30 = 0 mm, d3671_d952_d248_d13 = 0 mm, d3672_d953_d249_d14 = 0 mm, d3673_d954_d250_d15 = 270 deg, d3674_d955_d251_d16 = 0 mm, d3675_d956_d252_d17 = 270 deg, d3676_d957_d253_d3 = 25 deg, d3677_d958_d254_d4 = -25 deg, d3678_d959_d255_d5 = 25 deg, d3679_d960_d256_d6 = -25 deg, d3680_d961_d257_d2 = 0 mm, d3681_d962_d258_d30 = 0 mm, d3688_d952_d248_d13 = 0 mm, d3689_d953_d249_d14 = 0 mm, d3690_d954_d250_d15 = 270 deg, d3691_d955_d251_d16 = 0 mm, d3692_d956_d252_d17 = 270 deg, d3693_d957_d253_d3 = 25 deg, d3694_d958_d254_d4 = -25 deg, d3695_d959_d255_d5 = 25 deg, d3696_d960_d256_d6 = -25 deg, d3697_d961_d257_d2 = 0 mm, d3698_d962_d258_d30 = 0 mm